# Autodesk Inventor assembly: Vex Traction Wheel 6x1.5
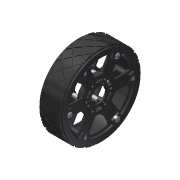
[picture p0: Inventor's stored thumbnail of the model, 180x180]
Saved by Autodesk Inventor 2013 (Build 170138000, 138)
## iProperties
Created: 2012-12-09
Part Number: Vex Traction Wheel 6x1.5
Document SubType Name: Assembly
Designer: Nemo
Author: Nemo
## Documents named in this file (7)
- H:\Nemo\Documents\Robotics\VexPro\Traction Wheel\Vex Traction Wheel 6x1.5.iam
- H:\Nemo\Documents\Robotics\VexPro\Traction Wheel\Components\Traction Tire Body 6in.ipt
- H:\Nemo\Documents\Robotics\VexPro\Fasteners\8-32 locknut.ipt
- H:\Nemo\Documents\Robotics\VexPro\Fasteners\Hex Standoff 8-32 x1250.ipt
- H:\Nemo\Documents\Robotics\VexPro\Fasteners\8-32 x1750 button head.ipt
- H:\Nemo\Documents\Robotics\VexPro\Traction Wheel\Components\Traction Tire extension 6in.ipt
- H:\Nemo\Documents\Robotics\VexPro\Traction Wheel\Components\6 Traction Tire - 1.5 Wide.ipt
## Components (22 placed, 6 different names)
1. Traction Tire Body 6in:1 — Mate:1, Mate:2, Angle:1, Insert:1, Insert:2, Angle:2, Insert:3, Mate:6, Mate:7
2. Traction Tire Body 6in:2 — Mate:3, Mate:4, Insert:4, Angle:3, Insert:5, Mate:8
3. Traction Tire extension 6in:1 — Mate:5, Mate:6, Mate:7, Mate:8, Mate:9
4. 6 Traction Tire - 1.5 Wide:1 — Mate:10, Mate:11, Mate:12
5. Hex Standoff 8-32 x1250:1 — Angle:1, Insert:1
6. Hex Standoff 8-32 x1250:2
7. Hex Standoff 8-32 x1250:3
8. Hex Standoff 8-32 x1250:4
9. Hex Standoff 8-32 x1250:5
10. Hex Standoff 8-32 x1250:6
11. 8-32 x1750 button head:1 — Insert:4
12. 8-32 locknut:2 — Angle:3, Insert:5
13. 8-32 x1750 button head:4 — Insert:3
14. 8-32 locknut:1 — Insert:2, Angle:2
15. 8-32 x1750 button head:2
16. 8-32 locknut:3
17. 8-32 x1750 button head:5
18. 8-32 locknut:4
19. 8-32 x1750 button head:3
20. 8-32 locknut:5
21. 8-32 x1750 button head:6
22. 8-32 locknut:6
## Component patterns: (6 elements, first: Hex Standoff 8-32 x1250:1), (3 elements, first: 8-32 x1750 button head:1 + 8-32 locknut:2 + 8-32 x1750 button head:4 + 8-32 locknut:1)
## Relationships (20: Mate 12, Insert 5, Angle 3)
- Mate:1: Traction Tire Body 6in:1
- Mate:2: Traction Tire Body 6in:1
- Angle:1 (0 deg): Traction Tire Body 6in:1 ↔ Hex Standoff 8-32 x1250:1
- Insert:1: Traction Tire Body 6in:1 ↔ Hex Standoff 8-32 x1250:1
- Insert:2: Traction Tire Body 6in:1 ↔ 8-32 locknut:1
- Angle:2 (0 deg): Traction Tire Body 6in:1 ↔ 8-32 locknut:1
- Insert:3: Traction Tire Body 6in:1 ↔ 8-32 x1750 button head:4
- Mate:3: Traction Tire Body 6in:2
- Mate:4: Traction Tire Body 6in:2
- Insert:4: Traction Tire Body 6in:2 ↔ 8-32 x1750 button head:1
- Angle:3 (0 deg): Traction Tire Body 6in:2 ↔ 8-32 locknut:2
- Insert:5: Traction Tire Body 6in:2 ↔ 8-32 locknut:2
- Mate:5: Traction Tire extension 6in:1
- Mate:6: Traction Tire Body 6in:1 ↔ Traction Tire extension 6in:1
- Mate:7: Traction Tire Body 6in:1 ↔ Traction Tire extension 6in:1
- Mate:8: Traction Tire Body 6in:2 ↔ Traction Tire extension 6in:1
- Mate:9: Traction Tire extension 6in:1
- Mate:10: 6 Traction Tire - 1.5 Wide:1
- Mate:11: 6 Traction Tire - 1.5 Wide:1
- Mate:12: 6 Traction Tire - 1.5 Wide:1
